# Autodesk Inventor assembly: Z Joint
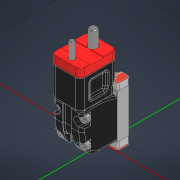
[picture p0: Inventor's stored thumbnail of the model, 180x180]
Saved by Autodesk Inventor 2022.2 (Build 262287010, 287A)
## iProperties
Created: 2022-03-14
Part Number: Z Joint
Document SubType Name: Assembly
Designer: sleib
Author: sleib
## Documents named in this file (10)
- C:\Users\sleib\Projekte\Voron-2\CAD\Inventor\Z Joint.iam
- C:\Users\sleib\Projekte\Voron-2\CAD\Inventor\MGN9H Carriage.ipt
- C:\Users\sleib\Projekte\Voron-2\CAD\Inventor\Z Bearing-Block Bottom.ipt
- C:\Users\sleib\Projekte\Voron-2\CAD\Inventor\Z Bearing-Block Top.ipt
- C:\Users\sleib\Projekte\Voron-2\CAD\Inventor\Z Belt-Clamp Lower.ipt
- C:\Users\sleib\Projekte\Voron-2\CAD\Inventor\M3x30 SHCS.ipt
- C:\Users\sleib\Projekte\Voron-2\CAD\Inventor\M3x20 SHCS.ipt
- C:\Users\sleib\Projekte\Voron-2\CAD\Inventor\M5 Hexnut.ipt
- C:\Users\sleib\Projekte\Voron-2\CAD\Inventor\M5x30 BHCS.ipt
- C:\Users\sleib\Projekte\Voron-2\CAD\Inventor\M5x40 SHCS.ipt
## Components (12 placed, 9 different names)
1. MGN9H Carriage:1 — Passend:1, Passend:2, Passend:3, Passend:4, Passend:13, Passend:14, Passend:15, Passend:16, Passend:17
2. Z Bearing-Block Bottom:1 — Passend:5, Passend:6, Passend:7, Passend:8, Passend:9, Passend:10, Passend:11, Passend:12, Passend:17, Tangential:1, Passend:29, Passend:30
3. Z Bearing-Block Top:1 — Passend:20, Passend:21, Passend:22, Passend:23, Tangential:1, Passend:28, Fluchtend:1, Passend:32, Winkel:1, Passend:33
4. Z Belt-Clamp Lower:1 — Passend:27, Passend:28, Fluchtend:1
5. M3x30 SHCS:1 — Passend:20, Passend:21
6. M3x20 SHCS:1 — Passend:5, Passend:10, Passend:13
7. M3x20 SHCS:2 — Passend:6, Passend:11, Passend:15
8. M3x20 SHCS:3 — Passend:7, Passend:9, Passend:16
9. M3x20 SHCS:4 — Passend:8, Passend:12, Passend:14
10. M5x30 BHCS:1 — Passend:22, Passend:23, Passend:27
11. M5x40 SHCS:1 — Passend:29, Passend:30, Passend:31, Passend:32
12. M5 Hexnut:1 — Passend:31, Winkel:1, Passend:33
## Relationships (31: Mate 28, Tangent 1, Flush 1, Angle 1)
- Passend:1 [Mate]: MGN9H Carriage:1
- Passend:2 [Mate]: MGN9H Carriage:1
- Passend:3 [Mate]: MGN9H Carriage:1
- Passend:4 [Mate]: MGN9H Carriage:1
- Passend:5 [Mate]: Z Bearing-Block Bottom:1 ↔ M3x20 SHCS:1
- Passend:6 [Mate]: Z Bearing-Block Bottom:1 ↔ M3x20 SHCS:2
- Passend:7 [Mate]: Z Bearing-Block Bottom:1 ↔ M3x20 SHCS:3
- Passend:8 [Mate]: Z Bearing-Block Bottom:1 ↔ M3x20 SHCS:4
- Passend:9 [Mate]: Z Bearing-Block Bottom:1 ↔ M3x20 SHCS:3
- Passend:10 [Mate]: Z Bearing-Block Bottom:1 ↔ M3x20 SHCS:1
- Passend:11 [Mate]: Z Bearing-Block Bottom:1 ↔ M3x20 SHCS:2
- Passend:12 [Mate]: Z Bearing-Block Bottom:1 ↔ M3x20 SHCS:4
- Passend:13 [Mate]: MGN9H Carriage:1 ↔ M3x20 SHCS:1
- Passend:14 [Mate]: MGN9H Carriage:1 ↔ M3x20 SHCS:4
- Passend:15 [Mate]: MGN9H Carriage:1 ↔ M3x20 SHCS:2
- Passend:16 [Mate]: MGN9H Carriage:1 ↔ M3x20 SHCS:3
- Passend:17 [Mate]: MGN9H Carriage:1 ↔ Z Bearing-Block Bottom:1
- Passend:20 [Mate]: Z Bearing-Block Top:1 ↔ M3x30 SHCS:1
- Passend:21 [Mate]: Z Bearing-Block Top:1 ↔ M3x30 SHCS:1
- Passend:22 [Mate]: Z Bearing-Block Top:1 ↔ M5x30 BHCS:1
- Passend:23 [Mate]: Z Bearing-Block Top:1 ↔ M5x30 BHCS:1
- Tangential:1: Z Bearing-Block Bottom:1 ↔ Z Bearing-Block Top:1
- Passend:27 [Mate]: Z Belt-Clamp Lower:1 ↔ M5x30 BHCS:1
- Passend:28 [Mate]: Z Bearing-Block Top:1 ↔ Z Belt-Clamp Lower:1
- Fluchtend:1 [Flush]: Z Bearing-Block Top:1 ↔ Z Belt-Clamp Lower:1
- Passend:29 [Mate]: Z Bearing-Block Bottom:1 ↔ M5x40 SHCS:1
- Passend:30 [Mate]: Z Bearing-Block Bottom:1 ↔ M5x40 SHCS:1
- Passend:31 [Mate]: M5x40 SHCS:1 ↔ M5 Hexnut:1
- Passend:32 [Mate]: Z Bearing-Block Top:1 ↔ M5x40 SHCS:1
- Winkel:1 [Angle] (0 deg): Z Bearing-Block Top:1 ↔ M5 Hexnut:1
- Passend:33 [Mate]: Z Bearing-Block Top:1 ↔ M5 Hexnut:1
